# Autodesk Inventor assembly: assembly of capping system
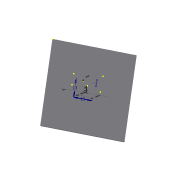
[picture p0: Inventor's stored thumbnail of the model, 180x180]
Saved by Autodesk Inventor 2019 (Build 230136000, 136)
## iProperties
Created: 2019-10-08
Part Number: assembly of capping system
Document SubType Name: Assembly
Designer: Admin
Author: Admin
## Documents named in this file (17)
- C:\Users\Admin\Documents\assembly of capping system.iam
- C:\Users\Admin\Documents\top support.ipt
- C:\Users\Admin\Documents\small nu 1.ipt
- C:\Users\Admin\Documents\dc motor.ipt
- C:\Users\Admin\Documents\lift dc motor.ipt
- C:\Users\Admin\Documents\bolt1.ipt
- C:\Users\Admin\Documents\dc motor nut.ipt
- C:\Users\Admin\Documents\nut1.ipt
- C:\Users\Admin\Documents\connector.ipt
- C:\Users\Admin\Documents\without head nut.ipt
- C:\Users\Admin\Documents\NUT SMALL.ipt
- C:\Users\Admin\Documents\SMP.ipt
- C:\Users\Admin\Documents\M.ipt
- C:\Users\Admin\Documents\ASSEMBLY DC MOTOR.iam
- C:\Users\Admin\Documents\CAPPER.ipt
- C:\Users\Admin\Documents\IR SENSOR ASSMBLY.iam
- C:\Users\Admin\Documents\base.ipt
## Components (27 placed, 16 different names)
1. top support:1 — Mate:1, Mate:2, Mate:3, Mate:4
2. small nu 1:1 — Mate:1, Mate:3, Mate:6, Rigid:1
3. small nu 1:2 — Mate:2, Mate:4, Mate:8, Rotational:1
4. dc motor:1 — Mate:5, Mate:7, Rotational:2, Mate:17, Mate:18
5. lift dc motor:1 — Mate:5, Mate:6, Mate:7, Mate:8, Mate:9, Mate:10, Rotational:3, Mate:11, Mate:12, Mate:13, Mate:14, Mate:15, Mate:16, Mate:44, Mate:45, Insert:7
6. bolt1:1 — Rigid:1, Rotational:3
7. bolt1:2 — Rotational:1
8. dc motor nut:1 — Rotational:2
9. nut1:1 — Mate:9, Mate:10
10. nut1:2 — Mate:11, Mate:14, Insert:4, Mate:43
11. nut1:3 — Mate:12, Mate:15, Insert:5, Mate:44, Mate:45
12. nut1:4 — Mate:13, Mate:16
13. connector:1 — Mate:17, Mate:18, Mate:19, Mate:28, Mate:29, Rotational:7, Mate:41, Mate:42, Rotational:11
14. without head nut:1 — Mate:19, Mate:28, Mate:29, Rotational:7, Rigid:2, Mate:41, Mate:42, Rotational:11, Rigid:4
15. NUT SMALL:1
16. NUT SMALL:2
17. bolt1:3 — Rigid:2
18. bolt1:4
19. bolt1:5
20. bolt1:6
21. SMP:1 — Insert:4, Insert:5, Rigid:5
22. M:1
23. ASSEMBLY DC MOTOR:1 [sub-assembly] — Rigid:4, Mate:43, Insert:6
24. CAPPER:1 — Insert:6
25. IR SENSOR ASSMBLY:1 [sub-assembly] — Rotational:12, Mate:46
26. base:1 — Rigid:5, Rotational:12, Mate:46
27. nut1:5 — Insert:7
## Relationships (41: Mate 27, RevoluteJoint 6, WeldJoint 4, Insert 4)
- Mate:1: top support:1 ↔ small nu 1:1
- Mate:2: top support:1 ↔ small nu 1:2
- Mate:3: top support:1 ↔ small nu 1:1
- Mate:4: top support:1 ↔ small nu 1:2
- Mate:5: dc motor:1 ↔ lift dc motor:1
- Mate:6: small nu 1:1 ↔ lift dc motor:1
- Mate:7: dc motor:1 ↔ lift dc motor:1
- Mate:8: small nu 1:2 ↔ lift dc motor:1
- Rigid:1 [WeldJoint]: small nu 1:1 ↔ bolt1:1
- Rotational:1 [RevoluteJoint]: small nu 1:2 ↔ bolt1:2
- Rotational:2 [RevoluteJoint]: dc motor:1 ↔ dc motor nut:1
- Mate:9: lift dc motor:1 ↔ nut1:1
- Mate:10: lift dc motor:1 ↔ nut1:1
- Rotational:3 [RevoluteJoint]: lift dc motor:1 ↔ bolt1:1
- Mate:11: lift dc motor:1 ↔ nut1:2
- Mate:12: lift dc motor:1 ↔ nut1:3
- Mate:13: lift dc motor:1 ↔ nut1:4
- Mate:14: lift dc motor:1 ↔ nut1:2
- Mate:15: lift dc motor:1 ↔ nut1:3
- Mate:16: lift dc motor:1 ↔ nut1:4
- Mate:17: dc motor:1 ↔ connector:1
- Mate:18: dc motor:1 ↔ connector:1
- Mate:19: connector:1 ↔ without head nut:1
- Mate:28: connector:1 ↔ without head nut:1
- Mate:29: connector:1 ↔ without head nut:1
- Rotational:7 [RevoluteJoint]: connector:1 ↔ without head nut:1
- Rigid:2 [WeldJoint] (25.4 mm): without head nut:1 ↔ bolt1:3
- Mate:41: connector:1 ↔ without head nut:1
- Mate:42: connector:1 ↔ without head nut:1
- Rotational:11 [RevoluteJoint]: connector:1 ↔ without head nut:1
- Insert:4: nut1:2 ↔ SMP:1
- Insert:5: nut1:3 ↔ SMP:1
- Rigid:4 [WeldJoint]: without head nut:1 ↔ ASSEMBLY DC MOTOR:1
- Mate:43: nut1:2 ↔ ASSEMBLY DC MOTOR:1
- Insert:6: ASSEMBLY DC MOTOR:1 ↔ CAPPER:1
- Mate:44: lift dc motor:1 ↔ nut1:3
- Mate:45: lift dc motor:1 ↔ nut1:3
- Rigid:5 [WeldJoint]: SMP:1 ↔ base:1
- Rotational:12 [RevoluteJoint]: IR SENSOR ASSMBLY:1 ↔ base:1
- Mate:46: IR SENSOR ASSMBLY:1 ↔ base:1
- Insert:7: lift dc motor:1 ↔ nut1:5
